# Autodesk Inventor assembly: Container_together
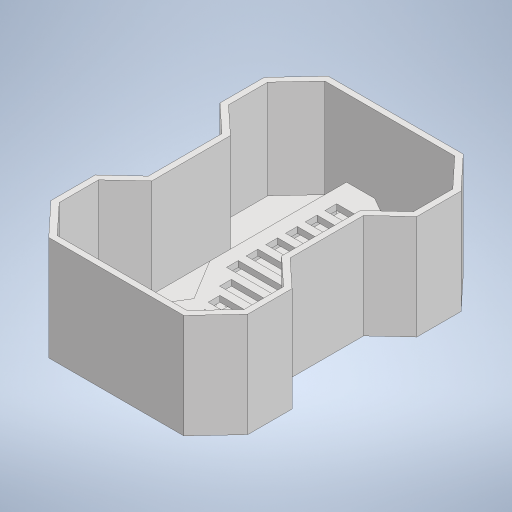
[picture p0: Inventor's stored thumbnail of the model, 512x512]
Saved by Autodesk Inventor 2024.2 (Build 282272000, 272)
## iProperties
Created: 2023-11-10
Part Number: Container_together
Document SubType Name: Assembly
Designer: Vincent
Author: Vincent
## Documents named in this file (5)
- D:\OneDrive - McMaster University\文档\School\1P13\Project 2\finalize_container\Container_together.iam
- D:\OneDrive - McMaster University\文档\School\1P13\Project 2\finalize_container\Container.ipt
- D:\OneDrive - McMaster University\文档\School\1P13\Project 2\finalize_container\Container_lid.ipt
- D:\OneDrive - McMaster University\文档\School\1P13\Project 2\Tool-2 (Bone Saw).ipt
- D:\OneDrive - McMaster University\文档\School\1P13\Project 2\Fooprint #1.ipt
## Components (4 placed, 4 different names)
1. Container:1 — Mate:1, Mate:2, Mate:3, Mate:4, Flush:1, Flush:2, Mate:5, Mate:6, Mate:7
2. Container_lid:1 — Mate:4, Flush:1, Flush:2
3. Tool-2 (Bone Saw):1 — Mate:1, Mate:2, Mate:3
4. Fooprint #1:1 — Mate:5, Mate:6, Mate:7
## Relationships (9: Mate 7, Flush 2)
- Mate:1: Container:1 ↔ Tool-2 (Bone Saw):1
- Mate:2 (2.5 mm): Container:1 ↔ Tool-2 (Bone Saw):1
- Mate:3 (2.5 mm): Container:1 ↔ Tool-2 (Bone Saw):1
- Mate:4: Container:1 ↔ Container_lid:1
- Flush:1: Container:1 ↔ Container_lid:1
- Flush:2: Container:1 ↔ Container_lid:1
- Mate:5: Container:1 ↔ Fooprint #1:1
- Mate:6 (1.5 mm): Container:1 ↔ Fooprint #1:1
- Mate:7 (12.5 mm): Container:1 ↔ Fooprint #1:1
